# Autodesk Inventor assembly: 15InVEX
(part 2 of 2)
- Flush:2: Alu C 1x2x1x29:3 ↔ 3rdAnd4thGearMount:1
- Flush:3: Alu C 1x2x1x29:3 ↔ 3rdAnd4thGearMount:1
- Flush:4: Alu C 1x2x1x29:3 ↔ 3rdAnd4thGearMount:1
- Insert:115: DriveGear2:3 ↔ Insert Square:5
- Insert:116: NSpacer Black .500 OD x .125:3 ↔ Insert Square:5
- Insert:117: NSpacer Black .500 OD x .125:3 ↔ TWasher .375 OD x .06250:8
- Tangent:2 (34.29 mm): DriveGear2:3 ↔ DriveGear2:4
- Flush:6: DriveGear2:3 ↔ DriveGear2:4
- Insert:119: 3rdAnd4thGearMount:1 ↔ DriveGear2:4
- Insert:120: DriveGear2:4 ↔ Insert Square:6
- Insert:121: NSpacer Black .500 OD x .125:4 ↔ Insert Square:6
- Insert:122: NSpacer Black .500 OD x .125:4 ↔ TWasher .375 OD x .06250:9
- Insert:123: Alu C 1x2x1x27:2 ↔ CombinedMotorMount:1
- Insert:124: Alu C 1x2x1x27:2 ↔ CombinedMotorMount:1
- Insert:125: DriveGear2:3 ↔ Insert Square:7
- Insert:126: DriveGear2:4 ↔ Insert Square:8
- Insert:127: 3rdAnd4thGearMount:1 ↔ Bearing Flat:3
- Insert:128: 3rdAnd4thGearMount:1 ↔ Bearing Flat:3
- Insert:129: 3rdAnd4thGearMount:1 ↔ Bearing Flat:4
- Insert:130: 3rdAnd4thGearMount:1 ↔ Bearing Flat:4
- Insert:131: NSpacer Black .500 OD x .125:6 ↔ Insert Square:7
- Insert:132: NSpacer Black .500 OD x .125:7 ↔ Insert Square:8
- Insert:133: Bearing Flat:4 ↔ Nut Nylock:26
- Insert:134: Bearing Flat:4 ↔ Nut Nylock:27
- Insert:135: Bearing Flat:3 ↔ Nut Nylock:28
- Insert:136: Bearing Flat:3 ↔ Nut Nylock:29
- Insert:137: 3rdAnd4thGearMount:1 ↔ SScrew Star Smooth .875:21
- Insert:138: 3rdAnd4thGearMount:1 ↔ SScrew Star Smooth .875:22
- Insert:139: 3rdAnd4thGearMount:1 ↔ SScrew Star Smooth .875:23
- Insert:140: 3rdAnd4thGearMount:1 ↔ SScrew Star Smooth .875:24
- Insert:141: Alu C 1x3x1x29:1 ↔ Nut Nylock:30
- Insert:144: Alu C 1x3x1x29:1 ↔ SScrew Star Smooth 1.750:25
- Insert:145: Alu C 1x2x1x29:3 ↔ SScrew Star Smooth 1.750:26
- Insert:146: Alu C 1x2x1x29:3 ↔ SScrew Star Smooth 1.500:27
- Insert:147: Alu C 1x2x1x29:3 ↔ Nut Nylock:36
- Insert:148: Alu C 1x2x1x29:3 ↔ Nut Nylock:37
- Insert:149: Alu C 1x2x1x29:3 ↔ Nut Nylock:33
- Insert:150: Alu C 1x2x1x29:3 ↔ Nut Nylock:34
- Insert:151: Alu C 1x2x1x29:3 ↔ Nut Nylock:35
- Insert:152: Alu C 1x2x1x29:3 ↔ Nut Nylock:38
- Insert:153: DriveGear2:4 ↔ SScrew Star Smooth .250:28
- Insert:154: DriveGear2:3 ↔ SScrew Star Smooth .250:29
- Insert:155: Alu C 1x3x1x29:1 ↔ SScrew Star Smooth 1.750:30
- Insert:156: Alu C 1x2x1x27:2 ↔ Nut Nylock:39
- Insert:157: Alu C 1x2x1x27:2 ↔ Nut Nylock:40
- Insert:158: CombinedMotorMount:1 ↔ SScrew Star Smooth 1.500:31
- Insert:159: CombinedMotorMount:1 ↔ SScrew Star Smooth 1.500:32
- Insert:160: Alu C 1x2x1x27:2 ↔ Nut Nylock:41
- Insert:161: Alu C 1x2x1x27:2 ↔ Nut Nylock:42
- Insert:162: Alu C 1x2x1x27:2 ↔ Nut Nylock:43
- Insert:163: Alu C 1x2x1x27:2 ↔ Nut Nylock:44
- Insert:164: Alu C 1x2x1x27:2 ↔ Nut Nylock:46
- Insert:165: Alu Angle 1x1x21:2 ↔ Nut Nylock:45
- Insert:166: Bearing Flat:2 ↔ Nut Nylock:47
- Insert:167: Bearing Flat:2 ↔ Nut Nylock:48
- Insert:168: Alu C 1x2x1x29:3 ↔ SScrew Star Smooth .500:33
- Insert:169: Alu C 1x2x1x29:3 ↔ SScrew Star Smooth .500:34
- Insert:170: 3rdAnd4thGearMount:1 ↔ Shaft LS 3.5:2
- Insert:171: 3rdAnd4thGearMount:1 ↔ Shaft LS 3.5:4
- Insert:172: Bearing Flat:1 ↔ Shaft LS 3.5:3
- Insert:173: Alu C 1x2x1x27:1 ↔ SScrew Star Smooth 2.000:46
- Insert:174: Alu C 1x2x1x27:1 ↔ Nut Thin Nylock:13
- Insert:175: Alu C 1x2x1x27:1 ↔ Nut Thin Nylock:14
- Insert:176: DriveGear1:4 ↔ 2.75 Omni AS, No Insert:4
- Insert:177: Alu C 1x2x1x27:1 ↔ TWasher .375 OD x .06250:10
- Insert:178: NSpacer Black .500 OD x .125:8 ↔ TWasher .375 OD x .06250:10
- Insert:179: 2.75 Omni AS, No Insert:4 ↔ Insert Circle:8
- Insert:180: Nut Nylock:49 ↔ Insert Circle:8
- Insert:181: TWasher .500 OD x .04000:11 ↔ Nut Nylock:49
- Insert:182: Alu C 1x2x1x29:5 ↔ Nut Nylock:50
- Insert:183: Bearing Flat:5 ↔ Nut Thin Nylock:16
- Insert:184: Bearing Flat:5 ↔ Nut Thin Nylock:15
- Insert:185: Alu C 1x2x1x29:5 ↔ Bearing Flat:5
- Insert:186: Alu C 1x2x1x29:5 ↔ Bearing Flat:5
- Insert:187: Alu C 1x2x1x29:5 ↔ Bearing Flat:6
- Insert:188: Alu C 1x2x1x29:5 ↔ Bearing Flat:6
- Insert:189: Alu C 1x2x1x29:5 ↔ SScrew Star Smooth .500:47
- Insert:190: Alu C 1x2x1x29:5 ↔ SScrew Star Smooth .500:48
- Insert:191: DriveGear2:5 ↔ Insert Square:9
- Insert:192: NSpacer .375 OD x .250:3 ↔ Insert Square:9
- Insert:193: NSpacer .375 OD x .250:3 ↔ TWasher .375 OD x .03125:12
- Insert:194: Alu C 1x2x1x27:1 ↔ TWasher .375 OD x .06250:13
- Insert:195: TWasher .375 OD x .06250:13 ↔ NSpacer Black .500 OD x .125:9
- Insert:196: DriveGear1:5 ↔ 2.75 Omni AS, No Insert:5
- Insert:197: DriveGear1:5 ↔ 2.75 Omni AS, No Insert:5
- Insert:198: DriveGear1:5 ↔ 2.75 Omni AS, No Insert:5
- Insert:199: DriveGear1:5 ↔ 2.75 Omni AS, No Insert:5
- Insert:200: DriveGear1:5 ↔ SScrew Star Smooth 1.000:49
- Insert:201: DriveGear1:5 ↔ SScrew Star Smooth 1.000:50
- Insert:202: DriveGear1:4 ↔ SScrew Star Smooth 1.000:51
- Insert:203: DriveGear1:4 ↔ SScrew Star Smooth 1.000:52
- Insert:204: Alu C 1x2x1x27:1 ↔ SScrew Star Smooth 2.000:53
- Insert:205: 2.75 Omni AS, No Insert:5 ↔ Insert Circle:9
- Insert:206: Nut Nylock:51 ↔ Insert Circle:9
- Insert:207: TWasher .500 OD x .04000:14 ↔ Nut Nylock:51
- Insert:208: Alu C 1x2x1x27:1 ↔ SScrew Star Smooth 2.000:55
- Insert:209: Alu C 1x2x1x27:1 ↔ Nut Thin Nylock:17
- Insert:210: DriveGear1:6 ↔ SScrew Star Smooth 1.000:54
- Insert:211: DriveGear1:6 ↔ SScrew Star Smooth 1.000:56
- Insert:212: DriveGear1:6 ↔ 2.75 Omni AS, No Insert:6
- Insert:213: DriveGear1:6 ↔ 2.75 Omni AS, No Insert:6
- Insert:214: DriveGear1:6 ↔ 2.75 Omni AS, No Insert:6
- Insert:215: 2.75 Omni AS, No Insert:4 ↔ Nut Thin Nylock:18
- Insert:216: 2.75 Omni AS, No Insert:4 ↔ Nut Thin Nylock:19
- Insert:217: 2.75 Omni AS, No Insert:5 ↔ Nut Thin Nylock:20
- Insert:218: 2.75 Omni AS, No Insert:5 ↔ Nut Thin Nylock:21
- Insert:219: 2.75 Omni AS, No Insert:6 ↔ Nut Thin Nylock:22
- Insert:220: 2.75 Omni AS, No Insert:6 ↔ Nut Thin Nylock:23
- Insert:221: DriveGear2:6 ↔ Insert Square:10
- Insert:222: NSpacer .375 OD x .250:4 ↔ Insert Square:10
- Insert:223: NSpacer .375 OD x .250:4 ↔ TWasher .375 OD x .03125:15
- Insert:224: 2.75 Omni AS, No Insert:6 ↔ Insert Circle:10
- Insert:225: Nut Nylock:52 ↔ Insert Circle:10
- Insert:226: TWasher .500 OD x .04000:16 ↔ Nut Nylock:52
- Insert:227: Alu C 1x2x1x29:5 ↔ Nut Nylock:53
- Insert:228: Alu C 1x2x1x29:5 ↔ Nut Nylock:54
- Insert:229: Alu C 1x2x1x27:1 ↔ CapOriginal:3
- Angle:3 (180 deg): Alu C 1x2x1x27:1 ↔ CapOriginal:3
- Insert:230: CapOriginal:3 ↔ SScrew Star Smooth 1.500:57
- Insert:231: CapOriginal:3 ↔ SScrew Star Smooth 1.500:58
- Insert:232: CapOriginal:3 ↔ SScrew Star Smooth 1.500:59
- Insert:233: Alu C 1x2x1x27:1 ↔ Nut Nylock:55
- Insert:234: Alu C 1x2x1x27:1 ↔ Nut Nylock:56
- Insert:235: Alu C 1x2x1x27:1 ↔ Nut Nylock:57
- Insert:236: CapOriginal:3 ↔ Nut Nylock:58
- Insert:237: Alu C 1x2x1x27:1 ↔ Nut Nylock:59
- Insert:238: Alu C 1x2x1x27:1 ↔ Nut Nylock:60
- Insert:239: CapOriginal:3 ↔ Nut Nylock:61
- Insert:240: CapOriginal:3 ↔ Nut Nylock:62
- Insert:241: Alu C 1x2x1x27:1 ↔ Nut Nylock:63
- Insert:243: Alu C 1x2x1x27:1 ↔ CapOriginal:4
- Insert:244: Alu C 1x2x1x27:1 ↔ CapOriginal:4
- Insert:245: CapOriginal:4 ↔ SScrew Star Smooth 1.500:60
- Insert:246: CapOriginal:4 ↔ SScrew Star Smooth 1.500:61
- Insert:247: CapOriginal:4 ↔ SScrew Star Smooth 1.500:62
- Insert:248: CapOriginal:4 ↔ Nut Nylock:64
- Insert:249: CapOriginal:4 ↔ Nut Nylock:65
- Insert:250: CapOriginal:4 ↔ Nut Nylock:66
- Insert:251: Alu C 1x2x1x27:1 ↔ Nut Nylock:67
- Insert:252: Alu C 1x2x1x27:1 ↔ Nut Nylock:68
- Insert:253: Alu C 1x2x1x27:1 ↔ Nut Nylock:69
- Insert:254: Alu C 1x2x1x27:1 ↔ Nut Nylock:70
- Insert:255: Alu C 1x2x1x27:1 ↔ Nut Nylock:71
- Insert:256: Alu C 1x2x1x27:1 ↔ Nut Nylock:72
- Flush:7: DriveGear2:5 ↔ DriveGear2:7
- Tangent:3 (34.29 mm): DriveGear2:5 ↔ DriveGear2:7
- Mate:4: Alu C 1x2x1x29:5 ↔ 3rdAnd4thGearMount_MIR:1
- Mate:5: Alu C 1x2x1x29:5 ↔ 3rdAnd4thGearMount_MIR:1
- Mate:6: Alu C 1x2x1x29:5 ↔ 3rdAnd4thGearMount_MIR:1
- Insert:257: NSpacer Black .500 OD x .125:10 ↔ TWasher .375 OD x .06250:17
- Flush:8: DriveGear2:7 ↔ DriveGear2:8
- Tangent:4 (34.29 mm): DriveGear2:7 ↔ DriveGear2:8
- Insert:259: NSpacer Black .500 OD x .125:11 ↔ TWasher .375 OD x .06250:18
- Insert:260: Alu C 1x2x1x27:1 ↔ CombinedMotorMount_MIR:1
- Insert:261: Alu C 1x2x1x27:1 ↔ CombinedMotorMount_MIR:1
- Insert:262: DriveGear2:7 ↔ Insert Square:11
- Insert:263: DriveGear2:8 ↔ Insert Square:12
- Insert:264: NSpacer Black .500 OD x .125:12 ↔ Insert Square:11
- Insert:265: 3rdAnd4thGearMount_MIR:1 ↔ Bearing Flat:7
- Insert:266: 3rdAnd4thGearMount_MIR:1 ↔ Bearing Flat:7
- Insert:267: 3rdAnd4thGearMount_MIR:1 ↔ Bearing Flat:8
- Insert:268: 3rdAnd4thGearMount_MIR:1 ↔ Bearing Flat:8
- Insert:269: NSpacer Black .500 OD x .125:13 ↔ Insert Square:12
- Insert:270: Bearing Flat:8 ↔ Nut Nylock:74
- Insert:271: Bearing Flat:8 ↔ Nut Nylock:75
- Insert:272: Bearing Flat:7 ↔ Nut Nylock:76
- Insert:273: Bearing Flat:7 ↔ Nut Nylock:77
- Insert:274: 3rdAnd4thGearMount_MIR:1 ↔ SScrew Star Smooth .875:35
- Insert:275: 3rdAnd4thGearMount_MIR:1 ↔ SScrew Star Smooth .875:36
- Insert:276: 3rdAnd4thGearMount_MIR:1 ↔ SScrew Star Smooth .875:37
- Insert:277: 3rdAnd4thGearMount_MIR:1 ↔ SScrew Star Smooth .875:38
- Insert:280: Alu C 1x2x1x29:5 ↔ SScrew Star Smooth 1.750:40
- Insert:281: Alu C 1x2x1x29:5 ↔ SScrew Star Smooth 1.500:41
- Insert:282: Alu C 1x2x1x29:5 ↔ Nut Nylock:81
- Insert:283: Alu C 1x2x1x29:5 ↔ Nut Nylock:82
- Insert:284: Alu C 1x2x1x29:5 ↔ Nut Nylock:83
- Insert:285: Alu C 1x2x1x29:5 ↔ Nut Nylock:84
- Insert:286: Alu C 1x2x1x29:5 ↔ Nut Nylock:85
- Insert:287: Alu C 1x2x1x29:5 ↔ Nut Nylock:86
- Insert:288: Alu C 1x2x1x27:1 ↔ Nut Nylock:87
- Insert:289: Alu C 1x2x1x27:1 ↔ Nut Nylock:88
- Insert:290: CombinedMotorMount_MIR:1 ↔ SScrew Star Smooth 1.500:43
- Insert:291: CombinedMotorMount_MIR:1 ↔ SScrew Star Smooth 1.500:44
- Insert:292: Alu C 1x2x1x27:1 ↔ Nut Nylock:89
- Insert:293: Alu C 1x2x1x27:1 ↔ Nut Nylock:90
- Insert:294: Alu C 1x2x1x27:1 ↔ Nut Nylock:91
- Insert:295: Alu C 1x2x1x27:1 ↔ Nut Nylock:92
- Insert:296: Alu Angle 1x1x21:2 ↔ Nut Nylock:93
- Insert:297: Alu C 1x2x1x27:1 ↔ Nut Nylock:94
- Insert:298: Bearing Flat:6 ↔ Nut Nylock:95
- Insert:299: Bearing Flat:6 ↔ Nut Nylock:96
- Insert:300: Alu C 1x2x1x29:5 ↔ SScrew Star Smooth .500:45
- Insert:301: Alu C 1x2x1x29:5 ↔ SScrew Star Smooth .500:63
- Insert:302: 3rdAnd4thGearMount_MIR:1 ↔ Shaft LS 3.5:6
- Insert:303: Bearing Flat:5 ↔ Shaft LS 3.5:7
- Insert:304: 3rdAnd4thGearMount_MIR:1 ↔ Shaft LS 3.5:8
- Insert:305: Alu C 1x3x1x29:1 ↔ Alu C 1x2x1x27:1
- Angle:4 (0 deg): Alu C 1x2x1x27:2 ↔ Alu C 1x2x1x27:1
- Insert:306: Alu C 1x3x1x29:1 ↔ Alu C 1x2x1x29:5
- Angle:5 (0 deg): Alu C 1x3x1x29:1 ↔ Alu C 1x2x1x29:5
- Insert:307: Alu C 1x2x1x29:5 ↔ 3rdAnd4thGearMount_MIR:1
- Insert:308: Alu C 1x2x1x27:1 ↔ CapOriginal:3
- Insert:309: DriveGear2:6 ↔ Insert Square:13
- Insert:310: DriveGear2:5 ↔ Insert Square:14
- Insert:311: DriveGear2:7 ↔ Insert Square:15
- Insert:312: NSpacer Black .500 OD x .125:9 ↔ Insert Square:13
- Insert:313: NSpacer Black .500 OD x .125:8 ↔ Insert Square:14
- Insert:314: Bearing Flat:7 ↔ NSpacer Black .500 OD x .125:12
- Insert:315: DriveGear2:8 ↔ Insert Square:16
- Insert:316: NSpacer Black .500 OD x .125:11 ↔ Insert Square:16
- Insert:317: DriveGear2:8 ↔ SScrew Star Smooth .250:65
- Insert:318: DriveGear2:7 ↔ SScrew Star Smooth .250:66
- Insert:319: DriveGear2:5 ↔ SScrew Star Smooth .250:64
- Insert:320: DriveGear2:6 ↔ SScrew Star Smooth .250:67
- Insert:321: Clamp:2 ↔ CapOriginal:3
- Angle:6 (0 deg): Clamp:2 ↔ CapOriginal:3
- Insert:322: Clamp:3 ↔ CapOriginal:4
- Angle:7 (0 deg): Clamp:3 ↔ CombinedMotorMount_MIR:1
- Insert:323: Clamp:4 ↔ CapOriginal:1
- Insert:324: Clamp:1 ↔ CapOriginal:2
- Mate:7: V5 Motor No Cap:1 ↔ CapOriginal:1
- Insert:325: V5 Motor No Cap:1 ↔ CapOriginal:1
- Mate:8: V5 Motor No Cap:2 ↔ CapOriginal:2
- Insert:326: V5 Motor No Cap:2 ↔ CapOriginal:2
- Mate:9: V5 Motor No Cap:3 ↔ CapOriginal:3
- Insert:327: V5 Motor No Cap:3 ↔ CapOriginal:3
- Mate:10: V5 Motor No Cap:4 ↔ CapOriginal:4
- Insert:328: V5 Motor No Cap:4 ↔ CapOriginal:4
- Insert:329: Bearing Flat:6 ↔ Shaft LS 3.5:10
- Insert:330: Bearing Flat:2 ↔ Shaft LS 3.5:9
- Insert:331: Alu Angle 1x1x21:1 ↔ Alu C 1x2x1x27:2
- Insert:332: Alu Angle 1x1x21:1 ↔ Alu C 1x2x1x27:1
- Insert:333: Alu Angle 1x1x21:2 ↔ Alu C 1x2x1x27:1
- Insert:334: Alu Angle 1x1x21:2 ↔ Alu C 1x2x1x27:2
- Insert:335: Alu Angle 1x1x21:1 ↔ SScrew Star Smooth 1.500:68
- Insert:336: Alu Angle 1x1x21:1 ↔ SScrew Star Smooth 1.500:69
- Insert:337: Alu C 1x2x1x27:1 ↔ Nut Nylock:98
- Insert:338: Alu C 1x2x1x27:1 ↔ Nut Nylock:97
- Insert:339: Alu C 1x2x1x27:1 ↔ Nut Nylock:99
- Insert:340: Alu C 1x2x1x27:2 ↔ Nut Nylock:102
- Insert:341: Alu C 1x2x1x27:2 ↔ Nut Nylock:101
- Insert:342: Alu C 1x2x1x27:2 ↔ Nut Nylock:100
- Insert:343: Alu C 1x2x1x21:1 ↔ Alu Angle 1x1x21:1
- Insert:344: Alu C 1x2x1x21:2 ↔ Alu Angle 1x1x21:1
- Insert:345: Alu C 1x2x1x21:2 ↔ Alu C 1x3x1x29:1
- Insert:346: Alu C 1x2x1x21:1 ↔ Alu C 1x3x1x29:1
- Mate:11: V5 Motor No Cap:6 ↔ CombinedMotorMount_MIR:1
- Insert:347: V5 Motor No Cap:6 ↔ CombinedMotorMount_MIR:1
- Angle:8 (0 deg): V5 Motor No Cap:6 ↔ CombinedMotorMount_MIR:1
- Mate:12: V5 Motor No Cap:5 ↔ CombinedMotorMount:1
- Insert:348: V5 Motor No Cap:5 ↔ CombinedMotorMount:1
- Angle:9 (180 deg): V5 Motor No Cap:5 ↔ CombinedMotorMount:1
- Insert:351: Alu C 1x2x1x21:2 ↔ Nut Nylock:103
- Insert:352: Alu C 1x2x1x21:1 ↔ Nut Nylock:104
- Insert:353: Alu C 1x2x1x21:2 ↔ Nut Nylock:106
- Insert:354: Alu C 1x2x1x21:2 ↔ Nut Nylock:107
- Insert:355: Alu C 1x2x1x21:1 ↔ Nut Nylock:105
- Insert:356: Alu C 1x2x1x21:1 ↔ Nut Nylock:108
- Insert:357: Alu Angle 1x1x21:2 ↔ SScrew Star Smooth 1.500:73
- Insert:358: Alu Angle 1x1x21:2 ↔ SScrew Star Smooth 1.500:72
- Insert:359: Alu C 1x2x1x21:2 ↔ Nut Nylock:114
- Insert:360: Alu C 1x2x1x21:2 ↔ Nut Nylock:110
- Insert:361: Alu C 1x2x1x21:1 ↔ Nut Nylock:109
- Insert:362: Alu C 1x2x1x21:1 ↔ Nut Nylock:112
- Insert:363: Alu C 1x2x1x21:1 ↔ Nut Nylock:111
- Insert:364: Alu C 1x2x1x21:2 ↔ Nut Nylock:113
- Insert:365: Alu C 1x3x1x29:1 ↔ SScrew Star Smooth 2.000:75
- Insert:366: Alu C 1x3x1x29:1 ↔ SScrew Star Smooth 2.000:74
- Insert:367: Alu C 1x2x1x21:2 ↔ Nut Nylock:115
- Insert:368: Alu C 1x2x1x21:2 ↔ Nut Nylock:116
- Insert:369: Alu C 1x3x1x29:1 ↔ Nut Nylock:117
- Insert:370: Alu C 1x3x1x29:1 ↔ Nut Nylock:119
- Insert:371: Alu C 1x3x1x29:1 ↔ Nut Nylock:120
- Insert:372: Alu C 1x2x1x21:1 ↔ Nut Nylock:118
- Insert:373: Alu C 1x2x1x21:1 ↔ Nut Nylock:121
- Insert:374: Alu C 1x3x1x29:1 ↔ Nut Nylock:122
- Insert:375: Alu C 1x2x1x21:2 ↔ NSpacer Black .500 OD x .125:15
- Insert:376: Alu C 1x2x1x21:1 ↔ NSpacer Black .500 OD x .125:14
- Insert:377: NSpacer Black .500 OD x .125:15 ↔ SWasher .375 OD x .031250:1
- Insert:378: NSpacer Black .500 OD x .125:14 ↔ SWasher .375 OD x .031250:2
- Mate:13: Funnel:1 ↔ Alu C 1x2x1x27:2
- Mate:14: Alu Angle 1x1x21:1 ↔ Funnel:1
- Mate:16: Funnel:1 ↔ Alu C 1x2x1x29:3
- Insert:413: Funnel:1 ↔ PolyRamp1:1
- Insert:414: SScrew Star Smooth .750:83 ↔ PolyRamp1:1
- Insert:417: Nut Nylock:137 ↔ Funnel_MIR:1
- Insert:418: Nut Nylock:139 ↔ Funnel_MIR:1
- Insert:419: Nut Nylock:138 ↔ Funnel:1
- Insert:420: Nut Nylock:140 ↔ Funnel:1
- Insert:421: Alu Angle 1x1x21:1 ↔ Ramp Support:1
- Insert:422: Alu Angle 1x1x21:1 ↔ Ramp Support:2
- Insert:423: SScrew Star Smooth .750:82 ↔ PolyRamp1:1
- Insert:424: SScrew Star Smooth .750:84 ↔ PolyRamp1:1
- Insert:425: SScrew Star Smooth .750:85 ↔ PolyRamp1:1
- Insert:428: SScrew Star Smooth .750:86 ↔ PolyRamp1:1
- Insert:429: SScrew Star Smooth .750:87 ↔ PolyRamp1:1
- Insert:430: Nut Nylock:142 ↔ Ramp Support:1
- Insert:432: SScrew Star Smooth 2.000:88 ↔ Ramp Support:1
- Insert:436: Alu Angle 1x1x21:1 ↔ Nut Nylock:143
- Insert:442: Alu C 1x2x1x29:5 ↔ Nut Nylock:145
- Insert:443: Alu C 1x2x1x29:5 ↔ Nut Nylock:146
- Insert:444: Alu C 1x2x1x29:5 ↔ Nut Nylock:148
- Insert:445: Alu C 1x2x1x29:5 ↔ Nut Nylock:152
- Insert:446: Alu C 1x2x1x29:5 ↔ Nut Nylock:151
- Insert:447: Alu C 1x2x1x29:5 ↔ Nut Nylock:153
- Insert:456: Alu C 1x2x1x29:3 ↔ Nut Nylock:157
- Insert:457: Alu C 1x2x1x29:3 ↔ Nut Nylock:154
- Insert:458: Alu C 1x2x1x29:3 ↔ Nut Nylock:156
- Insert:459: Alu C 1x2x1x29:3 ↔ Nut Nylock:155
- Insert:460: Nut Nylock:161 ↔ Alu C 1x2x1x29:3
- Insert:461: Alu C 1x2x1x29:3 ↔ Nut Nylock:159
- Insert:466: Alu Angle 1x1x21:1 ↔ Ramp Support:2
- Insert:467: SScrew Star Smooth 1.750:108 ↔ Ramp Support:2
- Insert:468: SScrew Star Smooth .875:109 ↔ Ramp Support:2
- Insert:469: SScrew Star Smooth .875:110 ↔ Ramp Support:1
- Insert:470: Alu Angle 1x1x21:1 ↔ Nut Nylock:162
- Insert:471: Nut Nylock:163 ↔ Ramp Support:2
- Rotation:1 [RelateRotation] (1 ul): DriveGear2:2 ↔ DriveGear1:3
- Rotation:2 [RelateRotation] (1 ul): DriveGear1:2 ↔ DriveGear2:2
- Rotation:3 [RelateRotation] (1 ul): DriveGear1:2 ↔ DriveGear2:1
- Rotation:4 [RelateRotation] (1 ul): DriveGear1:1 ↔ DriveGear2:1
- Rotation:5 [RelateRotation] (1 ul): DriveGear2:1 ↔ DriveGear2:3
- Rotation:6 [RelateRotation] (1 ul): DriveGear2:3 ↔ DriveGear2:4
- Insert:472: 3rdAnd4thGearMount:1 ↔ Nut Nylock:32
- Insert:473: Alu C 1x2x1x29:3 ↔ 3rdAnd4thGearMount:1
- Mate:17: V5 Motor No Cap:7 ↔ CombinedMotorMount:1
- Insert:474: V5 Motor No Cap:7 ↔ CombinedMotorMount:1
- Angle:10 (180 deg): V5 Motor No Cap:7 ↔ CombinedMotorMount:1
- Mate:18: V5 Motor No Cap:8 ↔ CombinedMotorMount_MIR:1
- Insert:475: V5 Motor No Cap:8 ↔ CombinedMotorMount_MIR:1
- Angle:11 (0 deg): V5 Motor No Cap:8 ↔ CombinedMotorMount_MIR:1
- Insert:476: Alu Angle 1x1x25:1 ↔ Alu C 1x2x1x21:1
- Flush:13: Alu C 1x2x1x21:1 ↔ AngleSupport:1
- Mate:19: Alu C 1x2x1x21:1 ↔ AngleSupport:1
- Mate:20: Alu C 1x2x1x21:1 ↔ AngleSupport:1
- Insert:477: Nut Nylock:164 ↔ AngleSupport:1
- Insert:478: Nut Nylock:165 ↔ AngleSupport:1
- Insert:479: Alu Angle 1x1x25:1 ↔ AngleSupport:1
- Insert:480: Alu Angle 1x1x25:1 ↔ AngleSupport:1
- Insert:481: Alu C 1x2x1x21:1 ↔ AngleSupport:1
- Insert:482: Alu C 1x2x1x21:1 ↔ AngleSupport:1
- Insert:483: Alu C 1x2x1x21:1 ↔ SScrew Star Smooth .750:112
- Insert:484: Alu C 1x2x1x21:1 ↔ SScrew Star Smooth .750:111
- Insert:485: Alu C 1x2x1x21:1 ↔ SScrew Star Smooth .750:113
- Insert:486: Nut Nylock:166 ↔ AngleSupport:1
- Insert:487: Nut Nylock:168 ↔ AngleSupport:1
- Insert:488: Nut Nylock:167 ↔ AngleSupport:1
- Insert:489: Alu Angle 1x1x25:1 ↔ SScrew Star Smooth .625:114
- Insert:490: Alu Angle 1x1x25:1 ↔ SScrew Star Smooth .625:115
- Insert:491: Alu Angle 1x1x25:2 ↔ Alu C 1x2x1x21:2
- Insert:492: Alu C 1x2x1x21:2 ↔ AngleSupport_MIR:1
- Insert:493: Alu C 1x2x1x21:2 ↔ AngleSupport_MIR:1
- Insert:494: Alu C 1x2x1x21:2 ↔ AngleSupport_MIR:1
- Insert:495: Alu Angle 1x1x25:2 ↔ AngleSupport_MIR:1
- Insert:496: Alu Angle 1x1x25:2 ↔ AngleSupport_MIR:1
- Insert:497: Alu Angle 1x1x25:2 ↔ SScrew Star Smooth .625:116
- Insert:498: Alu Angle 1x1x25:2 ↔ SScrew Star Smooth .625:117
- Insert:499: Nut Nylock:172 ↔ AngleSupport_MIR:1
- Insert:500: Nut Nylock:173 ↔ AngleSupport_MIR:1
- Insert:501: Nut Nylock:169 ↔ AngleSupport_MIR:1
- Insert:502: Nut Nylock:170 ↔ AngleSupport_MIR:1
- Insert:503: Nut Nylock:171 ↔ AngleSupport_MIR:1
- Insert:504: Alu C 1x2x1x21:2 ↔ SScrew Star Smooth .750:118
- Insert:505: Alu C 1x2x1x21:2 ↔ SScrew Star Smooth .750:119
- Insert:506: Alu C 1x2x1x21:2 ↔ SScrew Star Smooth .750:120
- Insert:507 (38.1 mm): Alu Angle 1x1x15:1 ↔ Alu Angle 1x1x25:1
- Angle:12 (180 deg): Alu Angle 1x1x15:1 ↔ Alu C 1x2x1x29:5
- Flush:14: IntakeSupport:1 ↔ Funnel_MIR:1
- Flush:15: IntakeSupport:1 ↔ Funnel_MIR:1
- Flush:16: IntakeSupport:1 ↔ Alu C 1x2x1x27:1
- Insert:509: IntakeSupport:1 ↔ Alu C 1x2x1x27:1
- Insert:510: IntakeSupport:1 ↔ Alu C 1x2x1x27:1
- Insert:514: Alu Angle 1x1x15:1 ↔ SScrew Star Smooth 2.000:121
- Insert:515: Alu Angle 1x1x15:1 ↔ Nut Nylock:176
- Insert:516: Alu Angle 1x1x25:1 ↔ Nut Nylock:175
- Insert:517: Alu Angle 1x1x25:1 ↔ Nut Nylock:174
- Insert:518: Nut Nylock:174 ↔ NSpacer White .500 OD x .500:16
- Insert:519: NSpacer White .500 OD x .500:16 ↔ NSpacer White .500 OD x .500:17
- Insert:520: NSpacer White .500 OD x .500:17 ↔ TWasher .500 OD x .04000:19
- Insert:525: Nut Nylock:177 ↔ Funnel_MIR:1
- Insert:526: Nut Nylock:178 ↔ Funnel_MIR:1
- Insert:527: Nut Nylock:179 ↔ Alu C 1x2x1x27:1
- Insert:528: Nut Nylock:180 ↔ Alu C 1x2x1x27:1
- Insert:529: NSpacer .375 OD x .500:5 ↔ Alu C 1x2x1x27:1
- Insert:530: NSpacer .375 OD x .500:6 ↔ Alu C 1x2x1x27:1
- Insert:531: NSpacer .375 OD x .500:6 ↔ NSpacer .375 OD x .375:7
- Insert:532: NSpacer .375 OD x .500:5 ↔ NSpacer .375 OD x .375:8
- Insert:535: Alu Angle 1x1x15:1 ↔ Nut Nylock:181
- Insert:536: Alu Angle 1x1x15:1 ↔ Nut Nylock:182
- Insert:537: Funnel_MIR:1 ↔ HardStop:2
- Insert:538: SScrew Star Smooth 1.500:124 ↔ IntakeSupport:1
- Insert:539: SScrew Star Smooth 1.500:122 ↔ IntakeSupport:1
- Insert:540: SScrew Star Smooth .750:126 ↔ IntakeSupport:1
- Insert:541: SScrew Star Smooth .750:127 ↔ IntakeSupport:1
- Insert:542: HardStop:3 ↔ Alu C 1x2x1x29:3
- Insert:543: HardStop:3 ↔ Funnel:1
- Insert:544: HardStop:3 ↔ SScrew Star Smooth 1.750:107
- Insert:545: HardStop:3 ↔ SScrew Star Smooth 1.750:105
- Insert:546: HardStop:3 ↔ SScrew Star Smooth 1.750:106
- Insert:547: HardStop:3 ↔ SScrew Star Smooth 1.750:104
- Insert:548: HardStop:2 ↔ SScrew Star Smooth 1.750:100
- Insert:549: HardStop:2 ↔ SScrew Star Smooth 1.750:101
- Insert:550: HardStop:2 ↔ SScrew Star Smooth 1.750:103
- Insert:551: HardStop:2 ↔ SScrew Star Smooth 1.750:102
- Insert:552: IntakeSupport_MIR:1 ↔ Funnel:1
- Insert:553: IntakeSupport_MIR:1 ↔ Funnel:1
- Insert:554: IntakeSupport_MIR:1 ↔ Alu C 1x2x1x27:2
- Insert:555: IntakeSupport_MIR:1 ↔ Alu C 1x2x1x27:2
- Insert:556 (38.1 mm): Alu Angle 1x1x15:2 ↔ Alu Angle 1x1x25:2
- Insert:557: Alu Angle 1x1x15:2 ↔ SScrew Star Smooth 2.000:128
- Insert:558: Alu Angle 1x1x25:2 ↔ Nut Nylock:183
- Insert:559: Alu Angle 1x1x15:2 ↔ Nut Nylock:184
- Insert:560: PolyIntakeSides:1 ↔ Nut Nylock:185
- Insert:561: Nut Nylock:184 ↔ NSpacer White .500 OD x .500:18
- Insert:562: NSpacer White .500 OD x .500:18 ↔ NSpacer White .500 OD x .500:19
- Insert:563: NSpacer White .500 OD x .500:19 ↔ TWasher .500 OD x .04000:20
- Insert:564: SScrew Star Smooth 1.500:129 ↔ IntakeSupport_MIR:1
- Insert:565: SScrew Star Smooth 1.500:130 ↔ IntakeSupport_MIR:1
- Insert:566: SScrew Star Smooth 1.500:131 ↔ IntakeSupport_MIR:1
- Insert:567: SScrew Star Smooth 1.500:132 ↔ IntakeSupport_MIR:1
- Insert:568: SScrew Star Smooth .750:133 ↔ IntakeSupport_MIR:1
- Insert:569: SScrew Star Smooth .750:134 ↔ IntakeSupport_MIR:1
- Insert:570: Alu Angle 1x1x15:2 ↔ Nut Nylock:186
- Insert:571: Alu Angle 1x1x15:2 ↔ Nut Nylock:187
- Insert:572: NSpacer .375 OD x .500:9 ↔ Alu C 1x2x1x27:2
- Insert:573: NSpacer .375 OD x .500:10 ↔ Alu C 1x2x1x27:2
- Insert:574: NSpacer .375 OD x .500:9 ↔ NSpacer .375 OD x .375:11
- Insert:575: NSpacer .375 OD x .500:10 ↔ NSpacer .375 OD x .375:12
- Insert:576: SScrew Star Smooth .375:135 ↔ Alu C 1x2x1x21:2
- Insert:577: SScrew Star Smooth .375:136 ↔ Alu C 1x2x1x21:2
- Insert:578: Nut Nylock:189 ↔ Funnel:1
- Insert:579: Nut Nylock:188 ↔ Funnel:1
- Angle:13 (0 deg): Alu Angle 1x1x15:2 ↔ Alu C 1x2x1x29:3
- Insert:582 (12.7 mm): Alu Angle 1x1x26:1 ↔ Alu Angle 1x1x15:2
- Flush:17 (-25.908 mm)
- Flush:18: TwistySupport:1 ↔ Alu Angle 1x1x25:2
- Flush:19: TwistySupport:1 ↔ Alu Angle 1x1x25:2
- Flush:20: Alu Angle 1x1x26:1 ↔ TwistySupport:1
- Insert:583: TwistySupport:1 ↔ Alu Angle 1x1x25:2
- Insert:584: Alu Angle 1x1x26:1 ↔ TwistySupport:1
- Insert:585: Alu Angle 1x1x26:1 ↔ TwistySupport:1
- Insert:586: Alu Angle 1x1x26:1 ↔ SScrew Star Smooth .750:137
- Insert:587: Alu Angle 1x1x26:1 ↔ SScrew Star Smooth .750:138
- Insert:588: TwistySupport:1 ↔ SScrew Star Smooth .750:139
- Insert:589: TwistySupport:1 ↔ SScrew Star Smooth .750:140
- Insert:590: TwistySupport:1 ↔ Nut Nylock:193
- Insert:591: Nut Nylock:192 ↔ PolyIntakeSides:1
- Insert:592: Nut Nylock:191 ↔ PolyIntakeSides:1
- Insert:593: TwistySupport:1 ↔ Nut Nylock:190
- Insert:598: Alu Angle 1x1x26:1 ↔ SScrew Star Smooth 2.500:141
- Insert:599: Alu Angle 1x1x26:1 ↔ Nut Nylock:194
- Insert:600: Nut Nylock:196 ↔ Alu Angle 1x1x15:2
- Insert:601: Nut Nylock:195 ↔ Alu Angle 1x1x15:2
- Insert:602: Nut Nylock:196 ↔ TWasher .500 OD x .04000:21
- Flush:21: PolyIntakeSides:1 ↔ Alu Angle 1x1x25:2
- Flush:22: PolyIntakeSides:1 ↔ Alu Angle 1x1x25:2
- Insert:611: SScrew Star Smooth 2.000:143 ↔ Alu Angle 1x1x15:2
- Insert:612: Nut Nylock:200 ↔ Alu Angle 1x1x15:2
- Insert:613: Nut Nylock:200 ↔ NSpacer .375 OD x .500:20
- Insert:614: NSpacer .375 OD x .500:18 ↔ NSpacer .375 OD x .500:20
- Insert:615: NSpacer .375 OD x .500:18 ↔ NSpacer .375 OD x .250:22
- Insert:616: NSpacer .375 OD x .250:22 ↔ TWasher .500 OD x .04000:23
- Insert:617: TWasher .500 OD x .04000:23 ↔ TWasher .500 OD x .04000:24
- Insert:618: PolyIntakeSides:1 ↔ Nut Nylock:201
- Flush:23 (38.1 mm): Alu C 1x2x1x21:2
- Insert:619: SScrew Star Smooth .375:144 ↔ Alu Angle 1x1x25:2
- Insert:620: PolyIntakeSides:1 ↔ Nut Nylock:202
- Insert:621: PolyIntakeSides:1 ↔ Nut Thin Nylock:24
- Insert:622: PolyIntakeSides:1 ↔ Nut Thin Nylock:25
- Insert:623: PolyIntakeSides:1 ↔ Nut Thin Nylock:26
- Insert:624: PolyIntakeSides:1 ↔ Nut Thin Nylock:27
- Insert:625: PolyIntakeSides:1 ↔ Nut Thin Nylock:28
- Insert:626: PolyIntakeSides:1 ↔ Nut Thin Nylock:29
- Insert:627: Standoff 4.00:5 ↔ Nut Thin Nylock:29
- Insert:628: Standoff 4.00:4 ↔ Nut Thin Nylock:28
- Insert:629: Standoff 4.00:3 ↔ Nut Thin Nylock:27
- Insert:630: Standoff 4.00:2 ↔ Nut Thin Nylock:26
- Insert:631: Standoff 4.00:1 ↔ Nut Thin Nylock:25
- Insert:632: Standoff 4.00:6 ↔ Nut Thin Nylock:24
- Insert:633: Standoff 4.00:5 ↔ Nut Thin Nylock:34
- Insert:634: Standoff 4.00:4 ↔ Nut Thin Nylock:35
- Insert:635: Standoff 4.00:3 ↔ Nut Thin Nylock:30
- Insert:636: Standoff 4.00:2 ↔ Nut Thin Nylock:31
- Insert:637: Standoff 4.00:6 ↔ Nut Thin Nylock:33
- Insert:638: Standoff 4.00:1 ↔ Nut Thin Nylock:32
- Insert:639: Nut Thin Nylock:33 ↔ PolyIntakeSides:2
- Insert:640: Nut Thin Nylock:32 ↔ PolyIntakeSides:2
- Insert:641: Nut Thin Nylock:31 ↔ PolyIntakeSides:2
- Insert:642: Nut Thin Nylock:30 ↔ PolyIntakeSides:2
- Insert:643: Nut Thin Nylock:35 ↔ PolyIntakeSides:2
- Insert:644: Nut Thin Nylock:34 ↔ PolyIntakeSides:2
- Flush:24: ChassisPolySides:1 ↔ Alu C 1x2x1x29:3
- Flush:25: ChassisPolySides:1 ↔ Alu C 1x2x1x29:3
- Insert:663: Standoff 1.50:7 ↔ CombinedMotorMount:1
- Insert:664: Standoff 1.50:8 ↔ CombinedMotorMount:1
- Insert:665: ChassisPolySides:1 ↔ SScrew Star Smooth 1.000:157
- Insert:666: ChassisPolySides:1 ↔ SScrew Star Smooth 1.000:158
- Insert:667: Standoff 1.50:7 ↔ Nut Nylock:203
- Insert:668: Standoff 1.50:8 ↔ Nut Nylock:204
- Insert:669: ChassisPolySides:1 ↔ Nut Nylock:206
- Insert:670: ChassisPolySides:1 ↔ Nut Nylock:205
- Insert:671: Nut Nylock:206 ↔ NSpacer .375 OD x .125:23
- Insert:672: Nut Nylock:205 ↔ NSpacer .375 OD x .125:24
- Insert:673: ChassisPolySides:1 ↔ SScrew Star Smooth 1.000:161
- Insert:674: ChassisPolySides:1 ↔ SScrew Star Smooth 1.000:159
- Insert:675: ChassisPolySides:1 ↔ SScrew Star Smooth 1.000:160
- Insert:676: ChassisPolySides:1 ↔ Standoff .50:10
- Insert:677: ChassisPolySides:1 ↔ Standoff .50:9
- Insert:678: ChassisPolySides:1 ↔ Standoff .50:11
- Insert:679: Nut Nylock:207 ↔ Alu C 1x2x1x29:3
- Insert:680: Nut Nylock:209 ↔ Alu C 1x2x1x29:3
- Insert:681: Nut Nylock:208 ↔ Alu C 1x2x1x29:3
- Insert:682 (12.7 mm): ChassisPolySides:2 ↔ Alu C 1x2x1x29:5
- Insert:683 (12.7 mm): ChassisPolySides:2 ↔ Alu C 1x2x1x29:5
- Insert:684 (12.7 mm): ChassisPolySides:2 ↔ Alu C 1x2x1x29:5
- Flush:26: PolyIntakeSides:2 ↔ Mesh:1
- Flush:27: PolyIntakeSides:2 ↔ Mesh:1
- Flush:28: BackPoly:1 ↔ Alu C 1x3x1x29:1
- Flush:29: BackPoly:1 ↔ Alu C 1x3x1x29:1
- Insert:685: BackPoly:1 ↔ SScrew Star Smooth .500:162
- Insert:688: BackPoly:1 ↔ SScrew Star Smooth .500:165
- Symmetry:1: ChassisPolySides:1 ↔ ChassisPolySides:2
- Insert:693: TwistySupport_MIR:1 ↔ Alu Angle 1x1x25:1
- Insert:694: TwistySupport_MIR:1 ↔ Alu Angle 1x1x25:1
- Insert:695: TwistySupport_MIR:1 ↔ Alu Angle 1x1x26:2
- Insert:696: TwistySupport_MIR:1 ↔ Alu Angle 1x1x26:2
- Insert:697 (38.1 mm): Poly3:1 ↔ Alu C 1x2x1x21:1
- Insert:698: Poly3:1 ↔ Alu C 1x2x1x21:2
- Insert:699: Poly3:1 ↔ Standoff 1.50:12
- Insert:700: Poly3:1 ↔ Standoff 1.50:14
- Insert:701: Poly3:1 ↔ Standoff 1.50:15
- Insert:702: Poly3:1 ↔ Standoff 1.50:13
- Insert:703: Poly3:1 ↔ SScrew Star Smooth .500:168
- Insert:704: Poly3:1 ↔ SScrew Star Smooth .500:166
- Insert:705: Poly3:1 ↔ SScrew Star Smooth .500:167
- Insert:706: Poly3:1 ↔ SScrew Star Smooth .500:169
- Insert:707: SScrew Star Smooth 1.500:170 ↔ Alu C 1x2x1x21:2
- Insert:708: SScrew Star Smooth 1.500:172 ↔ Alu C 1x2x1x21:1
- Insert:709: SScrew Star Smooth 1.500:173 ↔ Alu C 1x2x1x21:2
- Insert:710: SScrew Star Smooth 1.500:171 ↔ Alu C 1x2x1x21:1
- Insert:711: Nut Nylock:210 ↔ Alu C 1x2x1x21:1
- Insert:712: Nut Nylock:212 ↔ Alu C 1x2x1x21:1
- Insert:713: Nut Nylock:213 ↔ Alu C 1x2x1x21:1
- Insert:714: Nut Nylock:217 ↔ Alu C 1x2x1x21:1
- Insert:715: Nut Nylock:211 ↔ Alu C 1x2x1x21:2
- Insert:716: Nut Nylock:216 ↔ Alu C 1x2x1x21:2
- Insert:717: Nut Nylock:214 ↔ Alu C 1x2x1x21:2
- Insert:718: Nut Nylock:215 ↔ Alu C 1x2x1x21:2
- Insert:720: Alu Angle 1x1x26:2 ↔ SScrew Star Smooth 2.500:174
- Insert:721: Nut Nylock:218 ↔ Alu Angle 1x1x15:1
- Insert:722: Alu Angle 1x1x26:2 ↔ Nut Nylock:219
- Insert:723: Nut Nylock:220 ↔ Alu Angle 1x1x15:1
- Insert:726: Alu Angle 1x1x11:2 ↔ TWasher .500 OD x .04000:25
- Insert:727: RigidPieceFloat:1 ↔ Nut Thin Nylock:36
- Insert:728: RigidPieceFloat:1 ↔ SScrew Star Smooth .500:176
- Insert:729: RigidPieceFloat:1 ↔ SScrew Star Smooth .500:175
- Insert:730: Alu Angle 1x1x11:2 ↔ RigidPieceFloat:1
- Insert:731: Alu Angle 1x1x11:2 ↔ RigidPieceFloat:1
- Insert:732: Alu Angle 1x1x11:2 ↔ Nut Thin Nylock:37
- Insert:733: Alu Angle 1x1x11:2 ↔ Nut Thin Nylock:38
- Insert:736: Alu Angle 1x1x11:1 ↔ TWasher .500 OD x .04000:26
- Insert:737: Alu Angle 1x1x11:1 ↔ RigidPieceFloat:2
- Insert:738: Alu Angle 1x1x11:1 ↔ RigidPieceFloat:2
- Insert:739: RigidPieceFloat:2 ↔ SScrew Star Smooth .500:177
- Insert:740: RigidPieceFloat:2 ↔ SScrew Star Smooth .500:178
- Insert:741: RigidPieceFloat:2 ↔ TWasher .500 OD x .04000:27
- Insert:742: Nut Thin Nylock:41 ↔ TWasher .500 OD x .04000:27
- Insert:743: Alu Angle 1x1x11:1 ↔ Nut Thin Nylock:39
- Insert:744: Alu Angle 1x1x11:1 ↔ Nut Thin Nylock:40
- Flush:30: Alu Angle 1x1x11:1 ↔ OverTopRigidSup:1
- Flush:31: Alu Angle 1x1x11:1 ↔ OverTopRigidSup:1
- Insert:745: OverTopRigidSup:1 ↔ SScrew Star Smooth .500:179
- Insert:746: OverTopRigidSup:1 ↔ SScrew Star Smooth .500:180
- Insert:747: OverTopRigidSup:1 ↔ SScrew Star Smooth .500:181
- Insert:748: Alu Angle 1x1x11:1 ↔ Nut Nylock:221
- Insert:749: Alu Angle 1x1x11:1 ↔ Nut Nylock:222
- Insert:750: Alu Angle 1x1x11:1 ↔ Nut Nylock:223
- Insert:751: Alu Angle 1x1x11:2 ↔ OverTopRigidSup_MIR:1
- Insert:752: Alu Angle 1x1x11:2 ↔ OverTopRigidSup_MIR:1
- Angle:14 (0 deg): OverTopRigidSup:1 ↔ OverTopRigidSup_MIR:1
- Insert:753 (-5.08 mm): Alu Angle 1x1x11:2 ↔ Shaft HS 11.0 in:1
- Insert:754 (38.1 mm): Alu Angle 1x1x11:2 ↔ 1.625 30A .500:5
- Insert:755 (25.4 mm): 1.625 30A .500:5 ↔ 1.625 30A .500:6
- Insert:756 (25.4 mm): 1.625 30A .500:6 ↔ 1.625 30A .500:8
- Insert:757 (25.4 mm): 1.625 30A .500:3 ↔ 1.625 30A .500:8
- Insert:758 (25.4 mm): 1.625 30A .500:3 ↔ 1.625 30A .500:7
- Insert:759 (19.05 mm): 1.625 30A .500:4 ↔ 1.625 30A .500:7
- Insert:761: Alu Angle 1x1x11:2 ↔ HSpacer .1250:4
- Insert:763: HSpacer .1250:5 ↔ HS Shaft Collar:1
- Insert:764: HS Shaft Collar:1 ↔ HSpacer .2500:6
- Insert:765: 1.625 30A .500:5 ↔ HSpacer .5000:7
- Insert:766: 1.625 30A .500:6 ↔ HSpacer .5000:8
- Insert:767: 1.625 30A .500:6 ↔ HSpacer .5000:9
- Insert:768: HSpacer .5000:9 ↔ HSpacer .5000:10
- Insert:769: 1.625 30A .500:8 ↔ HSpacer .5000:11
- Insert:770: 1.625 30A .500:3 ↔ HSpacer .5000:12
- Insert:771: 1.625 30A .500:3 ↔ HSpacer .5000:13
- Insert:772: 1.625 30A .500:7 ↔ HSpacer .5000:15
- Insert:774: 1.625 30A .500:7 ↔ HSpacer .5000:16
- Insert:775: Alu Angle 1x1x11:1 ↔ HSpacer .1250:19
- Insert:776: HSpacer .1250:19 ↔ 9P 6T Sprocket, No Insert:7
- Insert:777: 9P 6T Sprocket, No Insert:7 ↔ HSpacer .1250:20
- Insert:778: HSpacer .1250:20 ↔ HS Shaft Collar:2
- Insert:779: HSpacer .5000:16 ↔ HSpacer .2500:21
- Insert:780: OverTopRigidSup:1 ↔ PolyIntakeTop:1
- Insert:781: OverTopRigidSup:1 ↔ PolyIntakeTop:1
- Insert:784: OverTopRigidSup:1 ↔ SScrew Star Smooth .500:184
- Insert:785: OverTopRigidSup:1 ↔ SScrew Star Smooth .500:185
- Insert:786: PolyIntakeTop:1 ↔ Nut Thin Nylock:42
- Insert:787: PolyIntakeTop:1 ↔ Nut Thin Nylock:43
- Insert:788: Alu Angle 1x1x11:1 ↔ Standoff 1.00:16
- Flush:32: Stage2:1 ↔ Alu Angle 1x1x15:2
- Flush:33: Stage2:1 ↔ Alu Angle 1x1x15:2
- Insert:791: Stage2:1 ↔ SScrew Star Smooth 1.500:188
- Insert:792: Stage2:1 ↔ SScrew Star Smooth 1.500:190
- Insert:793: Stage2:1 ↔ SScrew Star Smooth 1.500:191
- Insert:794: Nut Nylock:226 ↔ Alu Angle 1x1x15:2
- Insert:795: Nut Nylock:225 ↔ Alu Angle 1x1x15:2
- Insert:796: Nut Nylock:224 ↔ Alu Angle 1x1x15:2
- Insert:797: Nut Nylock:226 ↔ NSpacer Black .500 OD x .500:20
- Insert:798: Nut Nylock:225 ↔ NSpacer Black .500 OD x .500:21
- Insert:799: Nut Nylock:224 ↔ NSpacer Black .500 OD x .500:22
- Insert:806: Stage2:2 ↔ Nut Thin Nylock:46
- Insert:807: Stage2:2 ↔ Nut Thin Nylock:45
- Insert:808: Stage2:2 ↔ Nut Thin Nylock:44
- Insert:809: Stage2:2 ↔ SScrew Star Smooth 1.500:193
- Insert:810: Stage2:2 ↔ SScrew Star Smooth 1.500:192
- Insert:811: Stage2:2 ↔ NSpacer Black .500 OD x .500:20
- Insert:812: Stage2:2 ↔ NSpacer Black .500 OD x .500:21
- Insert:813: Stage2:1 ↔ Standoff .75:21
- Insert:814: Stage2:1 ↔ Standoff .75:22
- Insert:815: Standoff .75:21 ↔ TWasher .500 OD x .04000:28
- Insert:816: Standoff .75:22 ↔ TWasher .500 OD x .04000:29
- Insert:817: Stage2:1 ↔ HS Bearing Flat:1
- Insert:818: Stage2:1 ↔ HS Bearing Flat:1
- Insert:819: Stage2:2 ↔ Shaft HS 9.5 in:2
- Insert:821: Stage2:1 ↔ HSpacer .2500:22
- Insert:824: Stage2:1 ↔ Nut Nylock:229
- Insert:825: Stage2:1 ↔ Nut Nylock:230
- Insert:829: HSpacer .5000:24 ↔ HSpacer .1250:25
- Insert:832: Sprocket:1 ↔ HSpacer .0625:26
- Insert:833: Sprocket:1 ↔ HS Shaft Collar:4
- Insert:836: OdomHorizontal:1 ↔ Alu C 1x3x1x29:1
- Mate:21: DoubleOdom:1 ↔ Alu C 1x2x1x21:2
- Insert:837 (1.905 mm): HSpacer .2500:22 ↔ 6PSprocket:1
- Insert:839 (0.254 mm): HS Bearing Flat:1 ↔ 6PSprocket:2
- Insert:840: Nut Nylock:220 ↔ 6PSprocketElongated:1
- Insert:841 (0.381 mm): HSpacer .1250:4 ↔ 6PSprocket:3
- Insert:842: TWasher .500 OD x .04000:25 ↔ 6PSprocketElongated:2
- Insert:845: RoundyBit:1 ↔ Robert:1
- Insert:846: RoundyBit:1 ↔ Robert:1
- Insert:847: RoundyBit:1 ↔ Robert:1
- Insert:851: Robert_MIR:1 ↔ RoundyBit_MIR:1
- Insert:852: Robert_MIR:1 ↔ RoundyBit_MIR:1
- Insert:853: Alu Angle 1x1x26:2 ↔ PistonMech:1
- Insert:854: Alu Angle 1x1x26:1 ↔ PistonMech:1
- Insert:855: PistonMech:1 ↔ 25mm Stroke Pneumatic Cylinder:1
- Insert:856: RoundyBit_MIR:1 ↔ Alu Angle 1x1x25:2
- Insert:857: RoundyBit:1 ↔ Alu Angle 1x1x25:1
- Flush:34: Alu Angle 1x1x26:1 ↔ RoundFix:1
